# Autodesk Inventor assembly: Assembly1
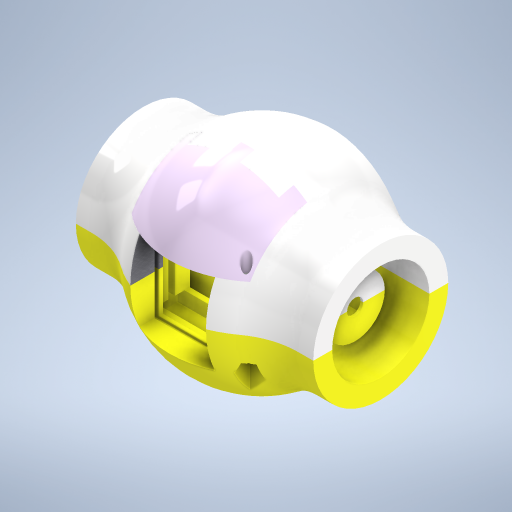
[picture p0: Inventor's stored thumbnail of the model, 512x512]
Saved by Autodesk Inventor 2023 (Build 270158000, 158)
## iProperties
Created: 2022-12-15
Part Number: Assembly1
Document SubType Name: Assembly
Designer: ellie
Author: ellie
## Documents named in this file (6)
- C:\Users\ellie\Documents\github\tanekonsat2022_runback\machinary\body\body back\back moter middle tire ver\Assembly1.iam
- C:\Users\ellie\Documents\github\tanekonsat2022_runback\machinary\body\body back\back moter middle tire ver\back moter middle lemon printing.ipt
- C:\Users\ellie\Documents\github\tanekonsat2022_runback\machinary\body\body back\back moter middle tire ver\back back printing2.ipt
- C:\Users\ellie\Documents\github\tanekonsat2022_runback\machinary\body\body front\front moter middle basic\body front moter middle lemon shape for printing.ipt
- C:\Users\ellie\Documents\github\tanekonsat2022_runback\machinary\parts\tire\tire out130 in 22 5mm inward.ipt
- C:\Users\ellie\Documents\github\tanekonsat2022_runback\machinary\parts\bush.ipt
## Components (7 placed, 4 different names)
1. body moter middle:1 — メイト:1, メイト:2, メイト:3, メイト:4, フラッシュ:1, メイト:5, メイト:6, メイト:7, メイト:8, メイト:9, メイト:10
2. body moter middle:2 — メイト:1, メイト:2
3. base front:1 — メイト:3, メイト:4, フラッシュ:1, メイト:11, メイト:12
4. tire out130 in 22 5mm inward:1 — メイト:5, メイト:6
5. tire out130 in 22 5mm inward:2 — メイト:7, メイト:8
6. bush:1 — メイト:11, メイト:12
7. bush:2 — メイト:9, メイト:10
## Relationships (13: Mate 12, Flush 1)
- メイト:1 [Mate]: body moter middle:1 ↔ body moter middle:2
- メイト:2 [Mate]: body moter middle:1 ↔ body moter middle:2
- メイト:3 [Mate]: body moter middle:1 ↔ base front:1
- メイト:4 [Mate]: body moter middle:1 ↔ base front:1
- フラッシュ:1 [Flush]: body moter middle:1 ↔ base front:1
- メイト:5 [Mate]: body moter middle:1 ↔ tire out130 in 22 5mm inward:1
- メイト:6 [Mate]: body moter middle:1 ↔ tire out130 in 22 5mm inward:1
- メイト:7 [Mate]: body moter middle:1 ↔ tire out130 in 22 5mm inward:2
- メイト:8 [Mate]: body moter middle:1 ↔ tire out130 in 22 5mm inward:2
- メイト:9 [Mate]: body moter middle:1 ↔ bush:2
- メイト:10 [Mate]: body moter middle:1 ↔ bush:2
- メイト:11 [Mate]: base front:1 ↔ bush:1
- メイト:12 [Mate]: base front:1 ↔ bush:1
